# Autodesk Inventor assembly: SlipRingAssy
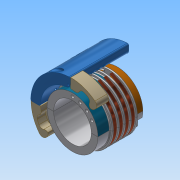
[picture p0: Inventor's stored thumbnail of the model, 180x180]
Saved by Autodesk Inventor 2017.3 (Build 213256000, 256)
## iProperties
Created: 2019-06-19
Part Number: SlipRingAssy
Document SubType Name: Assembly
Designer: Derek Wider
Author: Derek Wider
## Documents named in this file (7)
- G:\Projects\Submarine\Submarine-project\CAD\SlipRing\SlipRingAssy.iam
- G:\Projects\Submarine\Submarine-project\CAD\SlipRing\Core.ipt
- G:\Projects\Submarine\Submarine-project\CAD\SlipRing\CoreOpposite.ipt
- G:\Projects\Submarine\Submarine-project\CAD\SlipRing\BushingMount.ipt
- G:\Projects\Submarine\Submarine-project\CAD\SlipRing\ExtensionSpringSmall.ipt
- G:\Projects\Submarine\Submarine-project\CAD\SlipRing\BearingMount2.ipt
- G:\Projects\Submarine\Submarine-project\CAD\SlipRing\CopperContact.ipt
## Components (9 placed, 6 different names)
1. Core:1 — Mate:1, Mate:2, Flush:1, Mate:3, Angle:1, Flush:2, Mate:15, Mate:16
2. CoreOpposite:1 — Mate:1, Mate:2, Flush:1, Mate:7
3. BushingMount:1 — Mate:3, Angle:1, Mate:6, Flush:2, Mate:17
4. ExtensionSpringSmall:1 — Mate:6
5. BearingMount2:1 — Mate:7, Mate:17
6. CopperContact:1 — Mate:15, Mate:16
7. CopperContact:2
8. CopperContact:3
9. CopperContact:4
## Component patterns: (4 elements, first: CopperContact:1)
## Relationships (11: Mate 8, Flush 2, Angle 1)
- Mate:1: Core:1 ↔ CoreOpposite:1
- Mate:2: Core:1 ↔ CoreOpposite:1
- Flush:1: Core:1 ↔ CoreOpposite:1
- Mate:3: Core:1 ↔ BushingMount:1
- Angle:1 (0 deg): Core:1 ↔ BushingMount:1
- Mate:6: BushingMount:1 ↔ ExtensionSpringSmall:1
- Flush:2 (-1.778 mm): Core:1 ↔ BushingMount:1
- Mate:7: CoreOpposite:1 ↔ BearingMount2:1
- Mate:15: Core:1 ↔ CopperContact:1
- Mate:16 (0.8255 mm): Core:1 ↔ CopperContact:1
- Mate:17: BushingMount:1 ↔ BearingMount2:1
